# Autodesk Inventor assembly: 4005-0016-0001 Assembly Other Half
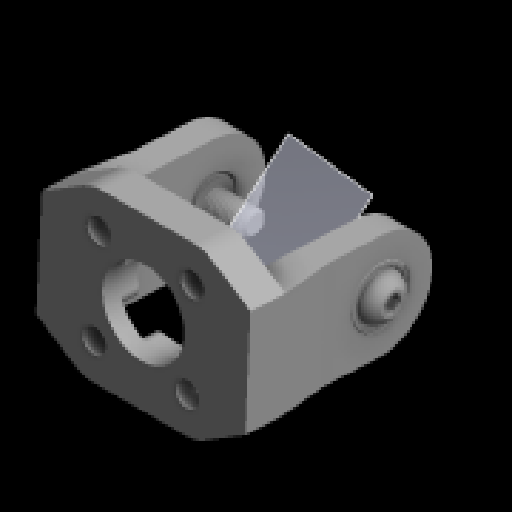
[picture p0: Inventor's stored thumbnail of the model, 512x512]
Saved by Autodesk Inventor 2025.2 (Build 292293000, 293)
## iProperties
Created: 2018-08-01
Part Number: 4005-0016-0001 Assembly Other Half
Description: STEP AP203
Document SubType Name: Assembly
Designer: valer
Sending System: SolidWorks 2016
Preprocessor: SwSTEP 2.0
Title: 4005-0016-0001 Assembly.STEP
Revision Number: ANY
## Documents named in this file (5)
- C:\Users\valer\Desktop\str1ker\cad\external\4005-0016-0001 Half.iam
- C:\Users\valer\Desktop\str1ker\cad\external\1600-0410-0004.ipt
- C:\Users\valer\Desktop\str1ker\cad\external\2802-0004-0012_92095A480.ipt
- C:\Users\valer\Desktop\str1ker\cad\external\2807-0407-1000.ipt
- C:\Users\valer\Desktop\str1ker\cad\external\4005-0016-0001 Outer Shell.ipt
## Components (7 placed, 7 different names)
1. 2807-0407-1000_6
2. 2807-0407-1000_8
3. 2802-0004-0012_92095A480_9
4. 2802-0004-0012_92095A480_11
5. 1600-0410-0004_12 — Symmetry:1
6. 1600-0410-0004_14 — Symmetry:1
7. 4005-0016-0001 Outer Shell_15
## Relationships (1: Symmetry 1)
- Symmetry:1: 1600-0410-0004_12 ↔ 1600-0410-0004_14
